# Autodesk Inventor assembly: 721114
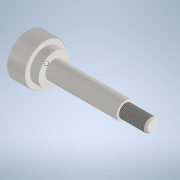
[picture p0: Inventor's stored thumbnail of the model, 180x180]
Saved by Autodesk Inventor 2022 (Build 260153000, 153)
## iProperties
Created: 2021-10-26
Part Number: 721114
Document SubType Name: Assembly
Designer: RaNSiD
Mass: 5717.92 g
Surface Area: 1100.13 cm^2
Volume: 728.397 cm^3
Density: 7.85 g/cm^3
Author: RaNSiD
## Documents named in this file (3)
- C:\Users\RaNSiD\Desktop\ВКР\Детали ЕСКД\721114.iam
- C:\Users\RaNSiD\Desktop\ВКР\Детали ЕСКД\721114 (Вал).ipt
- C:\Users\RaNSiD\Desktop\ВКР\Детали ЕСКД\721114\Мастер проектирования\Цилиндрическое зубчатое зацепление1.iam
## Components (2 placed, 2 different names)
1. 721114 (Вал) — Совмещение:1, Вставка:1
2. Цилиндрическое зубчатое зацепление:1 [sub-assembly] — Совмещение:1, Вставка:1
## Relationships (2: Mate 1, Insert 1)
- Совмещение:1 [Mate]: 721114 (Вал) ↔ Цилиндрическое зубчатое зацепление:1
- Вставка:1 [Insert]: 721114 (Вал) ↔ Цилиндрическое зубчатое зацепление:1
